# Autodesk Inventor assembly: Pergola
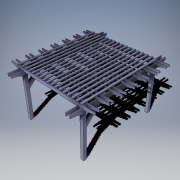
[picture p0: Inventor's stored thumbnail of the model, 180x180]
Saved by Autodesk Inventor 2016 (Build 200138000, 138)
## iProperties
Created: 2014-06-08
Part Number: Pergola
Document SubType Name: Assembly
Designer: Haden
Author: Haden
## Documents named in this file (6)
- C:\Users\Haden\Desktop\Desktop\CAD\Pergola\Pergola.iam
- C:\Users\Haden\Desktop\Desktop\CAD\Pergola\Post.ipt
- C:\Users\Haden\Desktop\Desktop\CAD\Pergola\Support Beam.ipt
- C:\Users\Haden\Desktop\Desktop\CAD\Pergola\Cover Board.ipt
- C:\Users\Haden\Desktop\Desktop\CAD\Pergola\Top Board.ipt
- C:\Users\Haden\Desktop\Desktop\CAD\Pergola\Angled Support.ipt
## Components (43 placed, 5 different names)
1. Post:1 — Flush:1, Flush:2, Flush:3, Flush:4, Flush:5, Flush:8, Flush:9, Mate:10, Mate:11, Flush:52
2. Post:2 — Flush:1, Flush:5, Flush:6, Flush:9
3. Post:3 — Flush:2, Flush:6, Flush:7, Mate:19
4. Post:4 — Flush:3, Flush:4, Flush:7, Flush:8, Mate:8, Mate:9, Flush:33, Mate:12, Mate:13, Flush:40, Flush:41, Mate:17, Flush:43, Flush:51, Mate:18
5. Support Beam:1 — Flush:27, Flush:30, Mate:8, Flush:33, Mate:16, Flush:53
6. Support Beam:2 — Flush:27, Flush:28, Flush:30, Flush:31, Mate:9
7. Support Beam:3 — Flush:28, Flush:29, Flush:31, Flush:32, Mate:10
8. Support Beam:4 — Flush:29, Flush:32, Mate:11
9. Angled Support:1 — Flush:44, Flush:46, Flush:48, Flush:49, Flush:51, Mate:18, Flush:53
10. Angled Support:2 — Flush:44, Flush:46, Flush:50, Flush:52
11. Angled Support:3 — Flush:45, Flush:47, Flush:48, Flush:49, Mate:19
12. Angled Support:4 — Flush:45, Flush:47, Flush:50
13. Cover Board:1 — Flush:34, Flush:37, Mate:12, Flush:40, Flush:41, Mate:16, Flush:42
14. Cover Board:2 — Flush:34, Flush:37, Mate:13
15. Cover Board:5
16. Cover Board:6
17. Cover Board:7
18. Cover Board:8
19. Cover Board:9
20. Cover Board:10
21. Cover Board:11
22. Cover Board:12
23. Cover Board:13
24. Cover Board:14
25. Cover Board:15
26. Cover Board:16
27. Top Board:1 — Mate:17, Flush:42, Flush:43
28. Top Board:2
29. Top Board:3
30. Top Board:4
31. Top Board:5
32. Top Board:6
33. Top Board:7
34. Top Board:8
35. Top Board:9
36. Top Board:10
37. Top Board:11
38. Top Board:12
39. Top Board:13
40. Top Board:14
41. Top Board:15
42. Top Board:16
43. Top Board:17
## Component patterns: (7 elements, first: Cover Board:1 + Cover Board:2), (17 elements, first: Top Board:1)
## Relationships (42: Flush 32, Mate 10)
- Flush:1: Post:1 ↔ Post:2
- Flush:2: Post:1 ↔ Post:3
- Flush:3: Post:1 ↔ Post:4
- Flush:4: Post:1 ↔ Post:4
- Flush:5: Post:1 ↔ Post:2
- Flush:6: Post:2 ↔ Post:3
- Flush:7: Post:3 ↔ Post:4
- Flush:8 (3048 mm): Post:1 ↔ Post:4
- Flush:9 (3657.6 mm): Post:1 ↔ Post:2
- Flush:27: Support Beam:1 ↔ Support Beam:2
- Flush:28: Support Beam:2 ↔ Support Beam:3
- Flush:29: Support Beam:3 ↔ Support Beam:4
- Flush:30: Support Beam:1 ↔ Support Beam:2
- Flush:31: Support Beam:2 ↔ Support Beam:3
- Flush:32: Support Beam:3 ↔ Support Beam:4
- Mate:8: Post:4 ↔ Support Beam:1
- Mate:9: Post:4 ↔ Support Beam:2
- Mate:10: Post:1 ↔ Support Beam:3
- Mate:11: Post:1 ↔ Support Beam:4
- Flush:33 (-539.75 mm): Post:4 ↔ Support Beam:1
- Flush:34: Cover Board:1 ↔ Cover Board:2
- Flush:37: Cover Board:1 ↔ Cover Board:2
- Mate:12: Post:4 ↔ Cover Board:1
- Mate:13: Post:4 ↔ Cover Board:2
- Flush:40: Post:4 ↔ Cover Board:1
- Flush:41: Post:4 ↔ Cover Board:1
- Mate:16: Support Beam:1 ↔ Cover Board:1
- Mate:17: Post:4 ↔ Top Board:1
- Flush:42: Cover Board:1 ↔ Top Board:1
- Flush:43: Post:4 ↔ Top Board:1
- Flush:44: Angled Support:1 ↔ Angled Support:2
- Flush:45: Angled Support:3 ↔ Angled Support:4
- Flush:46: Angled Support:1 ↔ Angled Support:2
- Flush:47: Angled Support:3 ↔ Angled Support:4
- Flush:48: Angled Support:1 ↔ Angled Support:3
- Flush:49: Angled Support:1 ↔ Angled Support:3
- Flush:50: Angled Support:2 ↔ Angled Support:4
- Flush:51: Post:4 ↔ Angled Support:1
- Flush:52: Post:1 ↔ Angled Support:2
- Mate:18: Post:4 ↔ Angled Support:1
- Mate:19: Post:3 ↔ Angled Support:3
- Flush:53: Support Beam:1 ↔ Angled Support:1
